# Autodesk Inventor assembly: Robot Assembly
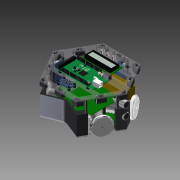
[picture p0: Inventor's stored thumbnail of the model, 180x180]
Saved by Autodesk Inventor 2015 (Build 190159000, 159)
## iProperties
Created: 2015-11-27
Part Number: Robot Assembly
Document SubType Name: Assembly
Designer: James
Mass: 1111.66 g
Surface Area: 2798.79 cm^2
Volume: 468.325 cm^3
Density: 2.3737 g/cm^3
Author: James
## Documents named in this file (26)
- C:\Users\James\Dropbox\Robotics 2016\Design\3D Printing\Version 2\Robot Assembly.iam
- C:\Users\James\Dropbox\Robotics 2016\Design\3D Printing\Version 2\Bottom Plate.ipt
- C:\Users\James\Dropbox\Robotics 2016\Design\3D Printing\Version 2\Support.ipt
- C:\Users\James\Dropbox\Robotics 2016\Design\3D Printing\Version 2\Front Support.ipt
- C:\Users\James\Dropbox\Robotics 2016\Design\3D Printing\Motor Mount Standoff.ipt
- C:\Users\James\Dropbox\Robotics 2016\Design\3D Printing\Motor Mount Bracket.ipt
- C:\Users\James\Dropbox\Robotics 2016\Design\3D Printing\Motor.ipt
- C:\Users\James\Dropbox\Robotics 2016\Design\3D Printing\Wheel.ipt
- C:\Users\James\Dropbox\Robotics 2016\Design\3D Printing\Spacer 5.ipt
- C:\Users\James\Dropbox\Robotics 2016\Design\3D Printing\Version 2\Bottom Plate Veroboard.ipt
- C:\Users\James\Dropbox\Robotics 2016\Design\3D Printing\Spacer 25.ipt
- C:\Users\James\Dropbox\Robotics 2016\Design\3D Printing\Version 2\Middle Plate Veroboard.ipt
- C:\Users\James\Dropbox\Robotics 2016\Design\3D Printing\M3 hex nut.ipt
- C:\Users\James\Dropbox\Robotics 2016\Design\3D Printing\Version 2\Top Plate.ipt
- C:\Users\James\Dropbox\Robotics 2016\Design\3D Printing\Version 2\TSOP Holder Straight.ipt
- C:\Users\James\Dropbox\Robotics 2016\Design\3D Printing\Version 2\TSOP Holder Corner.ipt
- C:\Users\James\Dropbox\Robotics 2016\Design\3D Printing\M3 6mm screw.ipt
- C:\Users\James\Dropbox\Robotics 2016\Design\3D Printing\ArduinoMEGA2560.ipt
- C:\Users\James\Dropbox\Robotics 2016\Design\3D Printing\lcd05-16x2.ipt
- C:\Users\James\Dropbox\Robotics 2016\Design\3D Printing\Adafruit Compass.ipt
- C:\Users\James\Dropbox\Robotics 2016\Design\3D Printing\LED Holder Nut.ipt
- C:\Users\James\Dropbox\Robotics 2016\Design\3D Printing\LED Holder.ipt
- C:\Users\James\Dropbox\Robotics 2016\Design\3D Printing\HC-SR04 Sonar.ipt
- C:\Users\James\Dropbox\Robotics 2016\Design\3D Printing\Back Support.ipt
- C:\Users\James\Dropbox\Robotics 2016\Design\3D Printing\M3 Metal Screw.ipt
- C:\Users\James\Dropbox\Robotics 2016\Design\3D Printing\Battery.ipt
## Components (163 placed, 25 different names)
1. Bottom Plate:1 — Mate:7, Mate:8, Mate:9, Mate:10, Mate:11, Mate:12, Mate:13, Mate:14, Mate:15, Mate:16, Mate:17, Mate:18, Mate:19, Mate:20, Mate:21, Mate:22, Mate:23, Mate:24, Mate:25, Mate:26, Mate:27, Mate:56, Mate:57, Mate:58, Mate:59, Mate:60, Mate:61, Mate:62, Mate:63, Mate:64, Mate:65, Mate:66, Mate:67, Mate:68, Mate:69, Mate:70, Mate:71, Mate:72, Mate:73, Mate:74, Mate:75, Mate:76, Mate:77, Mate:78, Mate:79, Mate:161, Mate:200, Mate:202, Mate:203, Mate:204, Mate:205, Mate:206, Mate:207, Mate:208, Mate:209, Mate:210, Mate:211, Mate:212, Mate:213, Mate:214, Mate:215, Mate:216, Mate:217, Mate:218, Mate:219, Mate:220, Mate:221, Mate:222, Mate:223, Mate:357, Mate:358, Mate:359, Mate:363, Mate:364, Mate:365, Mate:366, Mate:367, Mate:368, Mate:369, Mate:370, Mate:371, Mate:372, Mate:373, Mate:374, Mate:375, Mate:376, Mate:377, Mate:378, Mate:379, Mate:380, Mate:381, Mate:382, Mate:383, Mate:384, Mate:385, Mate:386, Mate:455
2. Support:1 — Mate:10, Mate:14, Mate:15, Mate:353, Mate:354, Mate:356
3. Support:2 — Mate:11, Mate:12, Mate:13, Mate:350, Mate:351, Mate:355
4. Front Support:1 — Mate:7, Mate:8, Mate:9, Mate:224, Mate:225, Mate:226
5. Motor Mount Standoff:1 — Mate:17, Mate:20, Mate:21, Mate:34, Mate:38, Mate:39
6. Motor Mount Standoff:2 — Mate:16, Mate:22, Mate:23, Mate:28, Mate:29, Mate:30
7. Motor Mount Standoff:3 — Mate:18, Mate:26, Mate:27, Mate:35, Mate:36, Mate:37
8. Motor Mount Standoff:4 — Mate:19, Mate:24, Mate:25, Mate:31, Mate:32, Mate:33
9. Motor Mount Bracket:1 — Mate:28, Mate:29, Mate:30, Mate:40, Mate:41, Mate:42
10. Motor Mount Bracket:2 — Mate:34, Mate:38, Mate:39, Mate:46, Mate:47, Mate:48
11. Motor Mount Bracket:3 — Mate:35, Mate:36, Mate:37, Mate:49, Mate:50, Mate:51
12. Motor Mount Bracket:4 — Mate:31, Mate:32, Mate:33, Mate:43, Mate:44, Mate:45
13. Motor:1 — Mate:40, Mate:41, Mate:42, Flush:4, Mate:55
14. Motor:2 — Mate:43, Mate:44, Mate:45, Flush:1, Mate:52
15. Motor:3 — Mate:46, Mate:47, Mate:48, Flush:3, Mate:54
16. Motor:4 — Mate:49, Mate:50, Mate:51, Flush:2, Mate:53
17. Wheel:1 — Flush:2, Mate:53
18. Wheel:2 — Flush:4, Mate:55
19. Wheel:3 — Flush:1, Mate:52
20. Wheel:4 — Flush:3, Mate:54
21. Spacer 5:1 — Mate:57, Mate:73, Mate:107
22. Spacer 5:2 — Mate:63, Mate:78, Mate:119
23. Spacer 5:3 — Mate:62, Mate:70, Mate:115
24. Spacer 5:4 — Mate:61, Mate:74, Mate:108
25. Spacer 5:5 — Mate:56, Mate:68, Mate:81, Mate:112
26. Spacer 5:6 — Mate:64, Mate:77, Mate:85
27. Spacer 5:7 — Mate:65, Mate:71, Mate:113
28. Spacer 5:8 — Mate:66, Mate:76, Mate:90
29. Spacer 5:9 — Mate:67, Mate:75, Mate:89
30. Spacer 5:10 — Mate:60, Mate:79, Mate:117
31. Spacer 5:11 — Mate:59, Mate:69, Mate:80, Mate:82, Mate:111
32. Spacer 5:12 — Mate:58, Mate:72, Mate:86
33. Bottom Plate Veroboard:1 — Mate:80, Mate:81, Mate:82, Mate:83, Mate:84, Mate:87, Mate:88, Mate:105, Mate:106, Mate:109, Mate:110, Mate:114, Mate:116, Mate:118, Mate:120
34. Spacer 25:1 — Mate:83, Mate:85, Mate:92, Mate:103
35. Spacer 25:2 — Mate:84, Mate:86, Mate:93, Mate:102
36. Spacer 25:3 — Mate:87, Mate:90, Mate:101
37. Spacer 25:4 — Mate:88, Mate:89, Mate:91, Mate:104
38. Middle Plate Veroboard:1 — Mate:91, Mate:92, Mate:93, Mate:94, Mate:95, Mate:96, Mate:100
39. M3 hex nut:1 — Mate:95, Mate:102
40. M3 hex nut:2 — Mate:96, Mate:101
41. M3 hex nut:3 — Mate:106, Mate:107
42. M3 hex nut:4 — Mate:94, Mate:104
43. M3 hex nut:5 — Mate:105, Mate:108
44. M3 hex nut:6 — Mate:100, Mate:103
45. M3 hex nut:11 — Mate:109, Mate:111
46. M3 hex nut:12 — Mate:113, Mate:114
47. M3 hex nut:13 — Mate:110, Mate:112
48. M3 hex nut:14 — Mate:117, Mate:118
49. M3 hex nut:15 — Mate:115, Mate:116
50. M3 hex nut:16 — Mate:119, Mate:120
51. TSOP Holder Straight:1 — Mate:233, Mate:234, Mate:235
52. TSOP Holder Straight:2 — Mate:227, Mate:228, Mate:229
53. TSOP Holder Straight:3 — Mate:239, Mate:240, Mate:241
54. TSOP Holder Straight:4 — Mate:257, Mate:258, Mate:259
55. TSOP Holder Straight:5 — Mate:245, Mate:246, Mate:247
56. TSOP Holder Straight:6 — Mate:251, Mate:252, Mate:253
57. TSOP Holder Corner:1 — Mate:254, Mate:255, Mate:256
58. TSOP Holder Corner:2 — Mate:242, Mate:243, Mate:244
59. TSOP Holder Corner:3 — Mate:236, Mate:237, Mate:238
60. TSOP Holder Corner:4 — Mate:248, Mate:249, Mate:250
61. TSOP Holder Corner:5 — Mate:230, Mate:231, Mate:232
62. TSOP Holder Corner:6 — Mate:260, Mate:261, Mate:262
63. M3 6mm screw:1 — Mate:209, Mate:217
64. M3 6mm screw:2 — Mate:211, Mate:219
65. M3 6mm screw:3 — Mate:213, Mate:221
66. M3 6mm screw:4 — Mate:203, Mate:207
67. M3 6mm screw:5 — Mate:210, Mate:216
68. M3 6mm screw:6 — Mate:212, Mate:220
69. M3 6mm screw:7 — Mate:161, Mate:206
70. M3 6mm screw:8 — Mate:214, Mate:222
71. M3 6mm screw:9 — Mate:215, Mate:223
72. M3 6mm screw:10 — Mate:208, Mate:218
73. M3 6mm screw:11 — Mate:200, Mate:204
74. M3 6mm screw:12 — Mate:202, Mate:205
75. -  -:1 — Mate:283, Mate:284, Mate:285, Mate:298, Mate:299, Mate:303, Mate:304, Mate:305, Mate:306, Mate:307, Mate:308, Mate:309, Mate:310, Mate:311, Mate:312
76. lcd05-16x2:1 — Mate:286, Mate:287, Mate:288
77. Adafruit Compass:1 — Mate:290, Mate:291, Mate:292, Mate:293, Mate:294, Mate:295, Mate:296, Mate:297, Mate:300, Mate:301, Mate:302
78. M3 6mm screw:13 — Mate:295, Mate:300
79. M3 6mm screw:14 — Mate:297, Mate:301
80. M3 6mm screw:15 — Mate:293, Mate:294
81. M3 6mm screw:16 — Mate:296, Mate:302
82. M3 6mm screw:17 — Mate:298, Mate:299
83. M3 6mm screw:18 — Mate:303, Mate:309
84. M3 6mm screw:19 — Mate:305, Mate:311
85. M3 6mm screw:20 — Mate:304, Mate:310
86. M3 6mm screw:21 — Mate:306, Mate:312
87. M3 6mm screw:22 — Mate:307, Mate:308
88. M3 hex nut:17 — Mate:347, Mate:348
89. M3 hex nut:18 — Mate:341, Mate:342
90. M3 hex nut:19 — Mate:331, Mate:332
91. M3 hex nut:20 — Mate:343, Mate:344
92. M3 hex nut:21 — Mate:345, Mate:346
93. M3 hex nut:22 — Mate:339, Mate:340
94. M3 hex nut:23 — Mate:335, Mate:336
95. M3 hex nut:24 — Mate:329, Mate:330
96. M3 hex nut:25 — Mate:333, Mate:334
97. M3 hex nut:26 — Mate:337, Mate:338
98. Spacer 5:13 — Mate:270, Mate:277, Mate:290, Mate:345
99. Spacer 5:14 — Mate:264, Mate:278, Mate:337
100. Spacer 5:15 — Mate:267, Mate:282, Mate:284, Mate:333
101. Spacer 5:16 — Mate:269, Mate:274, Mate:291, Mate:347
102. Spacer 5:17 — Mate:263, Mate:276, Mate:285, Mate:339
103. Spacer 5:18 — Mate:272, Mate:275, Mate:341
104. Spacer 5:19 — Mate:265, Mate:279, Mate:283, Mate:335
105. Spacer 5:20 — Mate:266, Mate:280, Mate:329
106. Spacer 5:21 — Mate:271, Mate:273, Mate:292, Mate:343
107. Spacer 5:22 — Mate:268, Mate:289, Mate:331
108. Top Plate:1 — Mate:224, Mate:225, Mate:226, Mate:227, Mate:228, Mate:229, Mate:230, Mate:231, Mate:232, Mate:233, Mate:234, Mate:235, Mate:236, Mate:237, Mate:238, Mate:239, Mate:240, Mate:241, Mate:242, Mate:243, Mate:244, Mate:245, Mate:246, Mate:247, Mate:248, Mate:249, Mate:250, Mate:251, Mate:252, Mate:253, Mate:254, Mate:255, Mate:256, Mate:257, Mate:258, Mate:259, Mate:260, Mate:261, Mate:262, Mate:263, Mate:264, Mate:265, Mate:266, Mate:267, Mate:268, Mate:269, Mate:270, Mate:271, Mate:272, Mate:273, Mate:274, Mate:275, Mate:276, Mate:277, Mate:278, Mate:279, Mate:280, Mate:282, Mate:286, Mate:287, Mate:288, Mate:289, Mate:313, Mate:314, Mate:315, Mate:317, Mate:318, Mate:320, Mate:321, Mate:322, Mate:324, Mate:330, Mate:332, Mate:334, Mate:336, Mate:338, Mate:340, Mate:342, Mate:344, Mate:346, Mate:348, Mate:387, Mate:388, Mate:389, Mate:390, Mate:391, Mate:392, Mate:393, Mate:394, Mate:395, Mate:396, Mate:397, Mate:398, Mate:399, Mate:400, Mate:401, Mate:402, Mate:403, Mate:404, Mate:405, Mate:407, Mate:408, Mate:409, Mate:410, Mate:411, Mate:412, Mate:413, Mate:415, Mate:416, Mate:417, Mate:418, Mate:419, Mate:420, Mate:421, Mate:422, Mate:423, Mate:424, Mate:425, Mate:426, Mate:427, Mate:428, Mate:429, Mate:430, Mate:431, Mate:432, Mate:433, Mate:434, Mate:435, Mate:436, Mate:437, Mate:438, Mate:439, Mate:440, Mate:441, Mate:442, Mate:443, Mate:444, Mate:445, Mate:446, Mate:447, Mate:448, Mate:449, Mate:450, Mate:451, Mate:452
109. LED Holder Nut:1 — Mate:323, Mate:324
110. LED Holder Nut:2 — Mate:319, Mate:320
111. LED Holder Nut:3 — Mate:315, Mate:316
112. LED Holder:1 — Mate:313, Mate:314, Mate:316
113. LED Holder:2 — Mate:317, Mate:318, Mate:319
114. LED Holder:3 — Mate:321, Mate:322, Mate:323
115. HC-SR04 Sonar:1 — Mate:350, Mate:351, Mate:355
116. HC-SR04 Sonar:2 — Mate:353, Mate:354, Mate:356
117. Back Support:1 — Mate:357, Mate:358, Mate:359, Mate:360, Mate:361, Mate:362, Mate:453, Mate:454, Flush:5
118. HC-SR04 Sonar:3 — Mate:360, Mate:361, Mate:362
119. M3 Metal Screw:1 — Mate:369, Mate:384
120. M3 Metal Screw:2 — Mate:368, Mate:383
121. M3 Metal Screw:3 — Mate:371, Mate:386
122. M3 Metal Screw:4 — Mate:370, Mate:385
123. M3 Metal Screw:5 — Mate:372, Mate:375
124. M3 Metal Screw:6 — Mate:373, Mate:376
125. M3 Metal Screw:7 — Mate:374, Mate:377
126. M3 Metal Screw:8 — Mate:363, Mate:378
127. M3 Metal Screw:9 — Mate:364, Mate:379
128. M3 Metal Screw:10 — Mate:367, Mate:380
129. M3 Metal Screw:11 — Mate:366, Mate:381
130. M3 Metal Screw:12 — Mate:365, Mate:382
131. M3 Metal Screw:13 — Mate:394, Mate:431
132. M3 Metal Screw:14 — Mate:395, Mate:434
133. M3 Metal Screw:15 — Mate:393, Mate:433
134. M3 Metal Screw:16 — Mate:392, Mate:419
135. M3 Metal Screw:17 — Mate:391, Mate:445
136. M3 Metal Screw:18 — Mate:387, Mate:443
137. M3 Metal Screw:19 — Mate:388, Mate:425
138. M3 Metal Screw:20 — Mate:389, Mate:422
139. M3 Metal Screw:21 — Mate:405, Mate:424
140. M3 Metal Screw:23 — Mate:413, Mate:442
141. M3 Metal Screw:24 — Mate:390, Mate:444
142. M3 Metal Screw:27 — Mate:415, Mate:441
143. M3 Metal Screw:28 — Mate:412, Mate:439
144. M3 Metal Screw:29 — Mate:411, Mate:437
145. M3 Metal Screw:30 — Mate:416, Mate:440
146. M3 Metal Screw:31 — Mate:410, Mate:438
147. M3 Metal Screw:32 — Mate:409, Mate:429
148. M3 Metal Screw:33 — Mate:408, Mate:432
149. M3 Metal Screw:34 — Mate:407, Mate:428
150. M3 Metal Screw:36 — Mate:404, Mate:426
151. M3 Metal Screw:37 — Mate:402, Mate:423
152. M3 Metal Screw:38 — Mate:403, Mate:427
153. M3 Metal Screw:39 — Mate:401, Mate:448
154. M3 Metal Screw:40 — Mate:399, Mate:430
155. M3 Metal Screw:41 — Mate:398, Mate:446
156. M3 Metal Screw:42 — Mate:400, Mate:447
157. M3 Metal Screw:43 — Mate:397, Mate:436
158. M3 Metal Screw:44 — Mate:396, Mate:435
159. M3 Metal Screw:45 — Mate:417, Mate:420
160. M3 Metal Screw:46 — Mate:418, Mate:421
161. M3 Metal Screw:47 — Mate:449, Mate:451
162. M3 Metal Screw:48 — Mate:450, Mate:452
163. Battery:1 — Mate:453, Mate:454, Flush:5
## Relationships (363: Mate 358, Flush 5)
- Mate:7: Bottom Plate:1 ↔ Front Support:1
- Mate:8: Bottom Plate:1 ↔ Front Support:1
- Mate:9: Bottom Plate:1 ↔ Front Support:1
- Mate:10: Bottom Plate:1 ↔ Support:1
- Mate:11: Bottom Plate:1 ↔ Support:2
- Mate:12: Bottom Plate:1 ↔ Support:2
- Mate:13: Bottom Plate:1 ↔ Support:2
- Mate:14: Bottom Plate:1 ↔ Support:1
- Mate:15: Bottom Plate:1 ↔ Support:1
- Mate:16: Bottom Plate:1 ↔ Motor Mount Standoff:2
- Mate:17: Bottom Plate:1 ↔ Motor Mount Standoff:1
- Mate:18: Bottom Plate:1 ↔ Motor Mount Standoff:3
- Mate:19: Bottom Plate:1 ↔ Motor Mount Standoff:4
- Mate:20: Bottom Plate:1 ↔ Motor Mount Standoff:1
- Mate:21: Bottom Plate:1 ↔ Motor Mount Standoff:1
- Mate:22: Bottom Plate:1 ↔ Motor Mount Standoff:2
- Mate:23: Bottom Plate:1 ↔ Motor Mount Standoff:2
- Mate:24: Bottom Plate:1 ↔ Motor Mount Standoff:4
- Mate:25: Bottom Plate:1 ↔ Motor Mount Standoff:4
- Mate:26: Bottom Plate:1 ↔ Motor Mount Standoff:3
- Mate:27: Bottom Plate:1 ↔ Motor Mount Standoff:3
- Mate:28: Motor Mount Standoff:2 ↔ Motor Mount Bracket:1
- Mate:29: Motor Mount Standoff:2 ↔ Motor Mount Bracket:1
- Mate:30: Motor Mount Standoff:2 ↔ Motor Mount Bracket:1
- Mate:31: Motor Mount Standoff:4 ↔ Motor Mount Bracket:4
- Mate:32: Motor Mount Standoff:4 ↔ Motor Mount Bracket:4
- Mate:33: Motor Mount Standoff:4 ↔ Motor Mount Bracket:4
- Mate:34: Motor Mount Standoff:1 ↔ Motor Mount Bracket:2
- Mate:35: Motor Mount Standoff:3 ↔ Motor Mount Bracket:3
- Mate:36: Motor Mount Standoff:3 ↔ Motor Mount Bracket:3
- Mate:37: Motor Mount Standoff:3 ↔ Motor Mount Bracket:3
- Mate:38: Motor Mount Standoff:1 ↔ Motor Mount Bracket:2
- Mate:39: Motor Mount Standoff:1 ↔ Motor Mount Bracket:2
- Mate:40: Motor Mount Bracket:1 ↔ Motor:1
- Mate:41: Motor Mount Bracket:1 ↔ Motor:1
- Mate:42: Motor Mount Bracket:1 ↔ Motor:1
- Mate:43: Motor Mount Bracket:4 ↔ Motor:2
- Mate:44: Motor Mount Bracket:4 ↔ Motor:2
- Mate:45: Motor Mount Bracket:4 ↔ Motor:2
- Mate:46: Motor Mount Bracket:2 ↔ Motor:3
- Mate:47: Motor Mount Bracket:2 ↔ Motor:3
- Mate:48: Motor Mount Bracket:2 ↔ Motor:3
- Mate:49: Motor Mount Bracket:3 ↔ Motor:4
- Mate:50: Motor Mount Bracket:3 ↔ Motor:4
- Mate:51: Motor Mount Bracket:3 ↔ Motor:4
- Flush:1: Motor:2 ↔ Wheel:3
- Mate:52: Motor:2 ↔ Wheel:3
- Flush:2: Motor:4 ↔ Wheel:1
- Mate:53: Motor:4 ↔ Wheel:1
- Flush:3: Motor:3 ↔ Wheel:4
- Mate:54: Motor:3 ↔ Wheel:4
- Flush:4: Motor:1 ↔ Wheel:2
- Mate:55: Motor:1 ↔ Wheel:2
- Mate:56: Bottom Plate:1 ↔ Spacer 5:5
- Mate:57: Bottom Plate:1 ↔ Spacer 5:1
- Mate:58: Bottom Plate:1 ↔ Spacer 5:12
- Mate:59: Bottom Plate:1 ↔ Spacer 5:11
- Mate:60: Bottom Plate:1 ↔ Spacer 5:10
- Mate:61: Bottom Plate:1 ↔ Spacer 5:4
- Mate:62: Bottom Plate:1 ↔ Spacer 5:3
- Mate:63: Bottom Plate:1 ↔ Spacer 5:2
- Mate:64: Bottom Plate:1 ↔ Spacer 5:6
- Mate:65: Bottom Plate:1 ↔ Spacer 5:7
- Mate:66: Bottom Plate:1 ↔ Spacer 5:8
- Mate:67: Bottom Plate:1 ↔ Spacer 5:9
- Mate:68: Bottom Plate:1 ↔ Spacer 5:5
- Mate:69: Bottom Plate:1 ↔ Spacer 5:11
- Mate:70: Bottom Plate:1 ↔ Spacer 5:3
- Mate:71: Bottom Plate:1 ↔ Spacer 5:7
- Mate:72: Bottom Plate:1 ↔ Spacer 5:12
- Mate:73: Bottom Plate:1 ↔ Spacer 5:1
- Mate:74: Bottom Plate:1 ↔ Spacer 5:4
- Mate:75: Bottom Plate:1 ↔ Spacer 5:9
- Mate:76: Bottom Plate:1 ↔ Spacer 5:8
- Mate:77: Bottom Plate:1 ↔ Spacer 5:6
- Mate:78: Bottom Plate:1 ↔ Spacer 5:2
- Mate:79: Bottom Plate:1 ↔ Spacer 5:10
- Mate:80: Spacer 5:11 ↔ Bottom Plate Veroboard:1
- Mate:81: Spacer 5:5 ↔ Bottom Plate Veroboard:1
- Mate:82: Spacer 5:11 ↔ Bottom Plate Veroboard:1
- Mate:83: Bottom Plate Veroboard:1 ↔ Spacer 25:1
- Mate:84: Bottom Plate Veroboard:1 ↔ Spacer 25:2
- Mate:85: Spacer 5:6 ↔ Spacer 25:1
- Mate:86: Spacer 5:12 ↔ Spacer 25:2
- Mate:87: Bottom Plate Veroboard:1 ↔ Spacer 25:3
- Mate:88: Bottom Plate Veroboard:1 ↔ Spacer 25:4
- Mate:89: Spacer 5:9 ↔ Spacer 25:4
- Mate:90: Spacer 5:8 ↔ Spacer 25:3
- Mate:91: Spacer 25:4 ↔ Middle Plate Veroboard:1
- Mate:92: Spacer 25:1 ↔ Middle Plate Veroboard:1
- Mate:93: Spacer 25:2 ↔ Middle Plate Veroboard:1
- Mate:94: Middle Plate Veroboard:1 ↔ M3 hex nut:4
- Mate:95: Middle Plate Veroboard:1 ↔ M3 hex nut:1
- Mate:96: Middle Plate Veroboard:1 ↔ M3 hex nut:2
- Mate:100: Middle Plate Veroboard:1 ↔ M3 hex nut:6
- Mate:101: Spacer 25:3 ↔ M3 hex nut:2
- Mate:102: Spacer 25:2 ↔ M3 hex nut:1
- Mate:103: Spacer 25:1 ↔ M3 hex nut:6
- Mate:104: Spacer 25:4 ↔ M3 hex nut:4
- Mate:105: Bottom Plate Veroboard:1 ↔ M3 hex nut:5
- Mate:106: Bottom Plate Veroboard:1 ↔ M3 hex nut:3
- Mate:107: Spacer 5:1 ↔ M3 hex nut:3
- Mate:108: Spacer 5:4 ↔ M3 hex nut:5
- Mate:109: Bottom Plate Veroboard:1 ↔ M3 hex nut:11
- Mate:110: Bottom Plate Veroboard:1 ↔ M3 hex nut:13
- Mate:111: Spacer 5:11 ↔ M3 hex nut:11
- Mate:112: Spacer 5:5 ↔ M3 hex nut:13
- Mate:113: Spacer 5:7 ↔ M3 hex nut:12
- Mate:114: Bottom Plate Veroboard:1 ↔ M3 hex nut:12
- Mate:115: Spacer 5:3 ↔ M3 hex nut:15
- Mate:116: Bottom Plate Veroboard:1 ↔ M3 hex nut:15
- Mate:117: Spacer 5:10 ↔ M3 hex nut:14
- Mate:118: Bottom Plate Veroboard:1 ↔ M3 hex nut:14
- Mate:119: Spacer 5:2 ↔ M3 hex nut:16
- Mate:120: Bottom Plate Veroboard:1 ↔ M3 hex nut:16
- Mate:161: Bottom Plate:1 ↔ M3 6mm screw:7
- Mate:200: Bottom Plate:1 ↔ M3 6mm screw:11
- Mate:202: Bottom Plate:1 ↔ M3 6mm screw:12
- Mate:203: Bottom Plate:1 ↔ M3 6mm screw:4
- Mate:204: Bottom Plate:1 ↔ M3 6mm screw:11
- Mate:205: Bottom Plate:1 ↔ M3 6mm screw:12
- Mate:206: Bottom Plate:1 ↔ M3 6mm screw:7
- Mate:207: Bottom Plate:1 ↔ M3 6mm screw:4
- Mate:208: Bottom Plate:1 ↔ M3 6mm screw:10
- Mate:209: Bottom Plate:1 ↔ M3 6mm screw:1
- Mate:210: Bottom Plate:1 ↔ M3 6mm screw:5
- Mate:211: Bottom Plate:1 ↔ M3 6mm screw:2
- Mate:212: Bottom Plate:1 ↔ M3 6mm screw:6
- Mate:213: Bottom Plate:1 ↔ M3 6mm screw:3
- Mate:214: Bottom Plate:1 ↔ M3 6mm screw:8
- Mate:215: Bottom Plate:1 ↔ M3 6mm screw:9
- Mate:216: Bottom Plate:1 ↔ M3 6mm screw:5
- Mate:217: Bottom Plate:1 ↔ M3 6mm screw:1
- Mate:218: Bottom Plate:1 ↔ M3 6mm screw:10
- Mate:219: Bottom Plate:1 ↔ M3 6mm screw:2
- Mate:220: Bottom Plate:1 ↔ M3 6mm screw:6
- Mate:221: Bottom Plate:1 ↔ M3 6mm screw:3
- Mate:222: Bottom Plate:1 ↔ M3 6mm screw:8
- Mate:223: Bottom Plate:1 ↔ M3 6mm screw:9
- Mate:224: Front Support:1 ↔ Top Plate:1
- Mate:225: Front Support:1 ↔ Top Plate:1
- Mate:226 (30 mm): Front Support:1 ↔ Top Plate:1
- Mate:227: TSOP Holder Straight:2 ↔ Top Plate:1
- Mate:228: TSOP Holder Straight:2 ↔ Top Plate:1
- Mate:229: TSOP Holder Straight:2 ↔ Top Plate:1
- Mate:230: TSOP Holder Corner:5 ↔ Top Plate:1
- Mate:231: TSOP Holder Corner:5 ↔ Top Plate:1
- Mate:232: TSOP Holder Corner:5 ↔ Top Plate:1
- Mate:233: TSOP Holder Straight:1 ↔ Top Plate:1
- Mate:234: TSOP Holder Straight:1 ↔ Top Plate:1
- Mate:235: TSOP Holder Straight:1 ↔ Top Plate:1
- Mate:236: TSOP Holder Corner:3 ↔ Top Plate:1
- Mate:237: TSOP Holder Corner:3 ↔ Top Plate:1
- Mate:238: TSOP Holder Corner:3 ↔ Top Plate:1
- Mate:239: TSOP Holder Straight:3 ↔ Top Plate:1
- Mate:240: TSOP Holder Straight:3 ↔ Top Plate:1
- Mate:241: TSOP Holder Straight:3 ↔ Top Plate:1
- Mate:242: TSOP Holder Corner:2 ↔ Top Plate:1
- Mate:243: TSOP Holder Corner:2 ↔ Top Plate:1
- Mate:244: TSOP Holder Corner:2 ↔ Top Plate:1
- Mate:245: TSOP Holder Straight:5 ↔ Top Plate:1
- Mate:246: TSOP Holder Straight:5 ↔ Top Plate:1
- Mate:247: TSOP Holder Straight:5 ↔ Top Plate:1
- Mate:248: TSOP Holder Corner:4 ↔ Top Plate:1
- Mate:249: TSOP Holder Corner:4 ↔ Top Plate:1
- Mate:250: TSOP Holder Corner:4 ↔ Top Plate:1
- Mate:251: TSOP Holder Straight:6 ↔ Top Plate:1
- Mate:252: TSOP Holder Straight:6 ↔ Top Plate:1
- Mate:253: TSOP Holder Straight:6 ↔ Top Plate:1
- Mate:254: TSOP Holder Corner:1 ↔ Top Plate:1
- Mate:255: TSOP Holder Corner:1 ↔ Top Plate:1
- Mate:256: TSOP Holder Corner:1 ↔ Top Plate:1
- Mate:257: TSOP Holder Straight:4 ↔ Top Plate:1
- Mate:258: TSOP Holder Straight:4 ↔ Top Plate:1
- Mate:259: TSOP Holder Straight:4 ↔ Top Plate:1
- Mate:260: TSOP Holder Corner:6 ↔ Top Plate:1
- Mate:261: TSOP Holder Corner:6 ↔ Top Plate:1
- Mate:262: TSOP Holder Corner:6 ↔ Top Plate:1
- Mate:263: Spacer 5:17 ↔ Top Plate:1
- Mate:264: Spacer 5:14 ↔ Top Plate:1
- Mate:265: Spacer 5:19 ↔ Top Plate:1
- Mate:266: Spacer 5:20 ↔ Top Plate:1
- Mate:267: Spacer 5:15 ↔ Top Plate:1
- Mate:268: Spacer 5:22 ↔ Top Plate:1
- Mate:269: Spacer 5:16 ↔ Top Plate:1
- Mate:270: Spacer 5:13 ↔ Top Plate:1
- Mate:271: Spacer 5:21 ↔ Top Plate:1
- Mate:272: Spacer 5:18 ↔ Top Plate:1
- Mate:273: Spacer 5:21 ↔ Top Plate:1
- Mate:274: Spacer 5:16 ↔ Top Plate:1
- Mate:275: Spacer 5:18 ↔ Top Plate:1
- Mate:276: Spacer 5:17 ↔ Top Plate:1
- Mate:277: Spacer 5:13 ↔ Top Plate:1
- Mate:278: Spacer 5:14 ↔ Top Plate:1
- Mate:279: Spacer 5:19 ↔ Top Plate:1
- Mate:280: Spacer 5:20 ↔ Top Plate:1
- Mate:282: Spacer 5:15 ↔ Top Plate:1
- Mate:283: -  -:1 ↔ Spacer 5:19
- Mate:284: -  -:1 ↔ Spacer 5:15
- Mate:285: -  -:1 ↔ Spacer 5:17
- Mate:286 (5 mm): lcd05-16x2:1 ↔ Top Plate:1
- Mate:287: lcd05-16x2:1 ↔ Top Plate:1
- Mate:288: lcd05-16x2:1 ↔ Top Plate:1
- Mate:289: Spacer 5:22 ↔ Top Plate:1
- Mate:290: Adafruit Compass:1 ↔ Spacer 5:13
- Mate:291: Adafruit Compass:1 ↔ Spacer 5:16
- Mate:292: Adafruit Compass:1 ↔ Spacer 5:21
- Mate:293: Adafruit Compass:1 ↔ M3 6mm screw:15
- Mate:294: Adafruit Compass:1 ↔ M3 6mm screw:15
- Mate:295: Adafruit Compass:1 ↔ M3 6mm screw:13
- Mate:296: Adafruit Compass:1 ↔ M3 6mm screw:16
- Mate:297: Adafruit Compass:1 ↔ M3 6mm screw:14
- Mate:298: -  -:1 ↔ M3 6mm screw:17
- Mate:299: -  -:1 ↔ M3 6mm screw:17
- Mate:300: Adafruit Compass:1 ↔ M3 6mm screw:13
- Mate:301: Adafruit Compass:1 ↔ M3 6mm screw:14
- Mate:302: Adafruit Compass:1 ↔ M3 6mm screw:16
- Mate:303: -  -:1 ↔ M3 6mm screw:18
- Mate:304: -  -:1 ↔ M3 6mm screw:20
- Mate:305: -  -:1 ↔ M3 6mm screw:19
- Mate:306: -  -:1 ↔ M3 6mm screw:21
- Mate:307: -  -:1 ↔ M3 6mm screw:22
- Mate:308: -  -:1 ↔ M3 6mm screw:22
- Mate:309: -  -:1 ↔ M3 6mm screw:18
- Mate:310: -  -:1 ↔ M3 6mm screw:20
- Mate:311: -  -:1 ↔ M3 6mm screw:19
- Mate:312: -  -:1 ↔ M3 6mm screw:21
- Mate:313: Top Plate:1 ↔ LED Holder:1
- Mate:314: Top Plate:1 ↔ LED Holder:1
- Mate:315: Top Plate:1 ↔ LED Holder Nut:3
- Mate:316: LED Holder Nut:3 ↔ LED Holder:1
- Mate:317: Top Plate:1 ↔ LED Holder:2
- Mate:318: Top Plate:1 ↔ LED Holder:2
- Mate:319: LED Holder Nut:2 ↔ LED Holder:2
- Mate:320: Top Plate:1 ↔ LED Holder Nut:2
- Mate:321: Top Plate:1 ↔ LED Holder:3
- Mate:322: Top Plate:1 ↔ LED Holder:3
- Mate:323: LED Holder Nut:1 ↔ LED Holder:3
- Mate:324: Top Plate:1 ↔ LED Holder Nut:1
- Mate:329: M3 hex nut:24 ↔ Spacer 5:20
- Mate:330: M3 hex nut:24 ↔ Top Plate:1
- Mate:331: M3 hex nut:19 ↔ Spacer 5:22
- Mate:332: M3 hex nut:19 ↔ Top Plate:1
- Mate:333: M3 hex nut:25 ↔ Spacer 5:15
- Mate:334: M3 hex nut:25 ↔ Top Plate:1
- Mate:335: M3 hex nut:23 ↔ Spacer 5:19
- Mate:336: M3 hex nut:23 ↔ Top Plate:1
- Mate:337: M3 hex nut:26 ↔ Spacer 5:14
- Mate:338: M3 hex nut:26 ↔ Top Plate:1
- Mate:339: M3 hex nut:22 ↔ Spacer 5:17
- Mate:340: M3 hex nut:22 ↔ Top Plate:1
- Mate:341: M3 hex nut:18 ↔ Spacer 5:18
- Mate:342: M3 hex nut:18 ↔ Top Plate:1
- Mate:343: M3 hex nut:20 ↔ Spacer 5:21
- Mate:344: M3 hex nut:20 ↔ Top Plate:1
- Mate:345: M3 hex nut:21 ↔ Spacer 5:13
- Mate:346: M3 hex nut:21 ↔ Top Plate:1
- Mate:347: M3 hex nut:17 ↔ Spacer 5:16
- Mate:348: M3 hex nut:17 ↔ Top Plate:1
- Mate:350: Support:2 ↔ HC-SR04 Sonar:1
- Mate:351: Support:2 ↔ HC-SR04 Sonar:1
- Mate:353: Support:1 ↔ HC-SR04 Sonar:2
- Mate:354: Support:1 ↔ HC-SR04 Sonar:2
- Mate:355: Support:2 ↔ HC-SR04 Sonar:1
- Mate:356: Support:1 ↔ HC-SR04 Sonar:2
- Mate:357: Bottom Plate:1 ↔ Back Support:1
- Mate:358: Bottom Plate:1 ↔ Back Support:1
- Mate:359: Bottom Plate:1 ↔ Back Support:1
- Mate:360: Back Support:1 ↔ HC-SR04 Sonar:3
- Mate:361: Back Support:1 ↔ HC-SR04 Sonar:3
- Mate:362: Back Support:1 ↔ HC-SR04 Sonar:3
- Mate:363: Bottom Plate:1 ↔ M3 Metal Screw:8
- Mate:364: Bottom Plate:1 ↔ M3 Metal Screw:9
- Mate:365: Bottom Plate:1 ↔ M3 Metal Screw:12
- Mate:366: Bottom Plate:1 ↔ M3 Metal Screw:11
- Mate:367: Bottom Plate:1 ↔ M3 Metal Screw:10
- Mate:368: Bottom Plate:1 ↔ M3 Metal Screw:2
- Mate:369: Bottom Plate:1 ↔ M3 Metal Screw:1
- Mate:370: Bottom Plate:1 ↔ M3 Metal Screw:4
- Mate:371: Bottom Plate:1 ↔ M3 Metal Screw:3
- Mate:372: Bottom Plate:1 ↔ M3 Metal Screw:5
- Mate:373: Bottom Plate:1 ↔ M3 Metal Screw:6
- Mate:374: Bottom Plate:1 ↔ M3 Metal Screw:7
- Mate:375: Bottom Plate:1 ↔ M3 Metal Screw:5
- Mate:376: Bottom Plate:1 ↔ M3 Metal Screw:6
- Mate:377: Bottom Plate:1 ↔ M3 Metal Screw:7
- Mate:378: Bottom Plate:1 ↔ M3 Metal Screw:8
- Mate:379: Bottom Plate:1 ↔ M3 Metal Screw:9
- Mate:380: Bottom Plate:1 ↔ M3 Metal Screw:10
- Mate:381: Bottom Plate:1 ↔ M3 Metal Screw:11
- Mate:382: Bottom Plate:1 ↔ M3 Metal Screw:12
- Mate:383: Bottom Plate:1 ↔ M3 Metal Screw:2
- Mate:384: Bottom Plate:1 ↔ M3 Metal Screw:1
- Mate:385: Bottom Plate:1 ↔ M3 Metal Screw:4
- Mate:386: Bottom Plate:1 ↔ M3 Metal Screw:3
- Mate:387: Top Plate:1 ↔ M3 Metal Screw:18
- Mate:388: Top Plate:1 ↔ M3 Metal Screw:19
- Mate:389: Top Plate:1 ↔ M3 Metal Screw:20
- Mate:390: Top Plate:1 ↔ M3 Metal Screw:24
- Mate:391: Top Plate:1 ↔ M3 Metal Screw:17
- Mate:392: Top Plate:1 ↔ M3 Metal Screw:16
- Mate:393: Top Plate:1 ↔ M3 Metal Screw:15
- Mate:394: Top Plate:1 ↔ M3 Metal Screw:13
- Mate:395: Top Plate:1 ↔ M3 Metal Screw:14
- Mate:396: Top Plate:1 ↔ M3 Metal Screw:44
- Mate:397: Top Plate:1 ↔ M3 Metal Screw:43
- Mate:398: Top Plate:1 ↔ M3 Metal Screw:41
- Mate:399: Top Plate:1 ↔ M3 Metal Screw:40
- Mate:400: Top Plate:1 ↔ M3 Metal Screw:42
- Mate:401: Top Plate:1 ↔ M3 Metal Screw:39
- Mate:402: Top Plate:1 ↔ M3 Metal Screw:37
- Mate:403: Top Plate:1 ↔ M3 Metal Screw:38
- Mate:404: Top Plate:1 ↔ M3 Metal Screw:36
- Mate:405: Top Plate:1 ↔ M3 Metal Screw:21
- Mate:407: Top Plate:1 ↔ M3 Metal Screw:34
- Mate:408: Top Plate:1 ↔ M3 Metal Screw:33
- Mate:409: Top Plate:1 ↔ M3 Metal Screw:32
- Mate:410: Top Plate:1 ↔ M3 Metal Screw:31
- Mate:411: Top Plate:1 ↔ M3 Metal Screw:29
- Mate:412: Top Plate:1 ↔ M3 Metal Screw:28
- Mate:413: Top Plate:1 ↔ M3 Metal Screw:23
- Mate:415: Top Plate:1 ↔ M3 Metal Screw:27
- Mate:416: Top Plate:1 ↔ M3 Metal Screw:30
- Mate:417: Top Plate:1 ↔ M3 Metal Screw:45
- Mate:418: Top Plate:1 ↔ M3 Metal Screw:46
- Mate:419: Top Plate:1 ↔ M3 Metal Screw:16
- Mate:420: Top Plate:1 ↔ M3 Metal Screw:45
- Mate:421: Top Plate:1 ↔ M3 Metal Screw:46
- Mate:422: Top Plate:1 ↔ M3 Metal Screw:20
- Mate:423: Top Plate:1 ↔ M3 Metal Screw:37
- Mate:424: Top Plate:1 ↔ M3 Metal Screw:21
- Mate:425: Top Plate:1 ↔ M3 Metal Screw:19
- Mate:426: Top Plate:1 ↔ M3 Metal Screw:36
- Mate:427: Top Plate:1 ↔ M3 Metal Screw:38
- Mate:428: Top Plate:1 ↔ M3 Metal Screw:34
- Mate:429: Top Plate:1 ↔ M3 Metal Screw:32
- Mate:430: Top Plate:1 ↔ M3 Metal Screw:40
- Mate:431: Top Plate:1 ↔ M3 Metal Screw:13
- Mate:432: Top Plate:1 ↔ M3 Metal Screw:33
- Mate:433: Top Plate:1 ↔ M3 Metal Screw:15
- Mate:434: Top Plate:1 ↔ M3 Metal Screw:14
- Mate:435: Top Plate:1 ↔ M3 Metal Screw:44
- Mate:436: Top Plate:1 ↔ M3 Metal Screw:43
- Mate:437: Top Plate:1 ↔ M3 Metal Screw:29
- Mate:438: Top Plate:1 ↔ M3 Metal Screw:31
- Mate:439: Top Plate:1 ↔ M3 Metal Screw:28
- Mate:440: Top Plate:1 ↔ M3 Metal Screw:30
- Mate:441: Top Plate:1 ↔ M3 Metal Screw:27
- Mate:442: Top Plate:1 ↔ M3 Metal Screw:23
- Mate:443: Top Plate:1 ↔ M3 Metal Screw:18
- Mate:444: Top Plate:1 ↔ M3 Metal Screw:24
- Mate:445: Top Plate:1 ↔ M3 Metal Screw:17
- Mate:446: Top Plate:1 ↔ M3 Metal Screw:41
- Mate:447: Top Plate:1 ↔ M3 Metal Screw:42
- Mate:448: Top Plate:1 ↔ M3 Metal Screw:39
- Mate:449: Top Plate:1 ↔ M3 Metal Screw:47
- Mate:450: Top Plate:1 ↔ M3 Metal Screw:48
- Mate:451: Top Plate:1 ↔ M3 Metal Screw:47
- Mate:452: Top Plate:1 ↔ M3 Metal Screw:48
- Mate:453: Back Support:1 ↔ Battery:1
- Mate:454 (10 mm): Back Support:1 ↔ Battery:1
- Flush:5 (24.195 mm): Back Support:1 ↔ Battery:1
- Mate:455 (5 mm): Bottom Plate:1
